# Autodesk Inventor assembly: AASTRC case
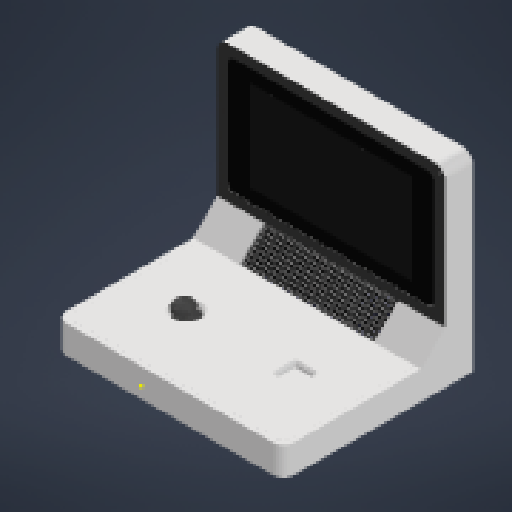
[picture p0: Inventor's stored thumbnail of the model, 512x512]
Saved by Autodesk Inventor 2024.2 (Build 282272000, 272)
## iProperties
Created: 2023-07-16
Part Number: AASTRC case
Document SubType Name: Assembly
Designer: 6gioc
Author: 6gioc
## Documents named in this file (8)
- C:\Users\6gioc\OneDrive\AAST\PART\AAST Remote Controler\AASTRC case.iam
- C:\Users\6gioc\OneDrive\AAST\PART\AAST Remote Controler\AASTRC Bottom case.ipt
- C:\Users\6gioc\OneDrive\AAST\PART\AAST Remote Controler\AASTRC Bottom case cover.ipt
- C:\Users\6gioc\OneDrive\AAST\PART\AAST Remote Controler\AASTRC Middle case cover assembly.iam
- C:\Users\6gioc\OneDrive\AAST\PART\AAST Remote Controler\AASTRC Top case cover.iam
- C:\Users\6gioc\OneDrive\AAST\PART\AAST Remote Controler\apple logo light module.iam
- C:\Users\6gioc\OneDrive\AAST\PART\AAST Remote Controler\KY-023_Joystick-Module\KY-023_Joystick-Module.iam
- C:\Users\6gioc\OneDrive\AAST\PART\AAST Remote Controler\KeySwitch.ipt
## Components (7 placed, 7 different names)
1. AASTRC Bottom case:1 — 강체:1, 강체:2, 강체:3, 강체:4, 강체:5, 강체:6
2. AASTRC Bottom case cover:1 — 강체:1
3. AASTRC Middle case cover assembly:1 [sub-assembly] — 강체:2
4. AASTRC Top case cover assemble:1 [sub-assembly] — 강체:3
5. apple logo light module:1 [sub-assembly] — 강체:4
6. KY-023_Joystick-Module:1 [sub-assembly] — 강체:5
7. KeySwitch:1 — 강체:6
## Relationships (6: WeldJoint 6)
- 강체:1 [WeldJoint]: AASTRC Bottom case:1 ↔ AASTRC Bottom case cover:1
- 강체:2 [WeldJoint]: AASTRC Bottom case:1 ↔ AASTRC Middle case cover assembly:1
- 강체:3 [WeldJoint]: AASTRC Bottom case:1 ↔ AASTRC Top case cover assemble:1
- 강체:4 [WeldJoint]: AASTRC Bottom case:1 ↔ apple logo light module:1
- 강체:5 [WeldJoint]: AASTRC Bottom case:1 ↔ KY-023_Joystick-Module:1
- 강체:6 [WeldJoint]: AASTRC Bottom case:1 ↔ KeySwitch:1
